# Autodesk Inventor assembly: Colson Performa 4x150
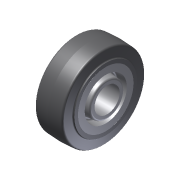
[picture p0: Inventor's stored thumbnail of the model, 180x180]
Saved by Autodesk Inventor 2013 (Build 170138000, 138)
## iProperties
Created: 2013-07-17
Part Number: Colson Performa 4x150
Document SubType Name: Assembly
Designer: Nemo
Author: Nemo
## Documents named in this file (3)
- H:\Nemo\Documents\Robotics\COTS Parts\Wheels\Colson Wheels\Colson Performa 4x150.iam
- H:\Nemo\Documents\Robotics\COTS Parts\Wheels\Colson Wheels\Components\Colson Performa Hub 4x150.ipt
- H:\Nemo\Documents\Robotics\COTS Parts\Wheels\Colson Wheels\Components\Colson Performa Tread 4x150.ipt
## Components (2 placed, 2 different names)
1. Colson Performa Hub 4x150:1 — Mate:1, Mate:2
2. Colson Performa Tread 4x150:1 — Mate:1, Mate:2
## Relationships (2: Mate 2)
- Mate:1: Colson Performa Hub 4x150:1 ↔ Colson Performa Tread 4x150:1
- Mate:2: Colson Performa Hub 4x150:1 ↔ Colson Performa Tread 4x150:1
